# Autodesk Inventor assembly: MX106T
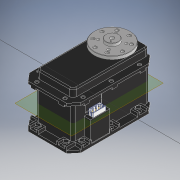
[picture p0: Inventor's stored thumbnail of the model, 180x180]
Saved by Autodesk Inventor 2022 (Build 260153000, 153)
## iProperties
Created: 2021-11-20
Part Number: MX106T
Description: STEP AP214
Document SubType Name: Assembly
Designer: Petrov Ivan
Sending System: SolidWorks 2016
Preprocessor: SwSTEP 2.0
Title: MX106T.STEP
Revision Number: ANY
## Documents named in this file (6)
- D:\IVAN\Ivan_desktop\Kvantorium\Projects\YouBotRobot\design\standart_components\dynamixels\mx-106\MX106T.iam
- D:\IVAN\Ivan_desktop\Kvantorium\Projects\YouBotRobot\design\standart_components\dynamixels\mx-106\MX-106T.ipt
- D:\IVAN\Ivan_desktop\Kvantorium\Projects\YouBotRobot\design\standart_components\dynamixels\mx-106\ROUE MX106T.ipt
- D:\IVAN\Ivan_desktop\Kvantorium\Projects\YouBotRobot\design\standart_components\dynamixels\mx-106\arbre MX106T.ipt
- D:\IVAN\Ivan_desktop\Kvantorium\Projects\YouBotRobot\design\standart_components\dynamixels\mx-106\Insert M3 à encastrer long 5mm.ipt
- D:\IVAN\Ivan_desktop\Kvantorium\Projects\YouBotRobot\design\standart_components\dynamixels\mx-106\connecteur dynamixel.ipt
## Components (6 placed, 6 different names)
1. MX-106T_1 — Совмещение:3, Угол:1
2. ROUE MX106T_2 — Совмещение:1, Совмещение:2
3. arbre MX106T_3 — Совмещение:1, Совмещение:2
4. Insert M3 à encastrer long 5mm_4
5. connecteur dynamixel_5
6. connecteur dynamixel_6
## Relationships (4: Mate 3, Angle 1)
- Совмещение:1 [Mate]: ROUE MX106T_2 ↔ arbre MX106T_3
- Совмещение:2 [Mate]: ROUE MX106T_2 ↔ arbre MX106T_3
- Совмещение:3 [Mate]: MX-106T_1
- Угол:1 [Angle] (0 deg): MX-106T_1
